# Autodesk Inventor assembly: 043(F,D-166-3)
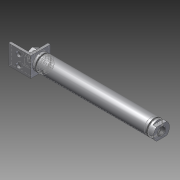
[picture p0: Inventor's stored thumbnail of the model, 180x180]
Saved by Autodesk Inventor 2012 (Build 160160000, 160)
## iProperties
Category: PARTsolutions
Company: BIMBA
Created: 2013-01-17
Part Number: 043(F,D-166-3)
Catalog Web Link: www.cadenas.de
Description: Original Line Standard Air Cylinders-
Vendor: BIMBA
Document SubType Name: Assembly
Designer: William
Manufacturer: BIMBA
PSOL_IDENT_0: {\\10.0.0.242\data_v9\23d-libs\bimba\bimba\bimba_imperial\bimba_full_line\original_line_cylinders\st
PSOL_IDENT_1: andard_air_cylinders\standard_air_cylinder_asmtab.prj},308 {VTYP=3D},{STYP=ASSTAB},{NB=043(F,D-166-3
PSOL_IDENT_2: )},{LINA=043},{NN=Original Line Standard Air Cylinders},{DATE=06.09.2012 11:26:56},{GEOMDATE=06.09.2
PSOL_IDENT_3: 012},{VERSION=},{LINEID=50},{LINESUBID=-1},{WBVAR=STROKE,ACTING,MNT,DER,NR,BM,CO,OO,VO,M,EE,EEL,K,Q,
PSOL_IDENT_4: Y,G,T,B,H,SER,SR,NT,W,HL,STPT1,STPT2,STPT3,STPT4,MB,PB,PRC,TB,MN}  {NB=043(F,D-166-3)},{LINA=043},{K
PSOL_IDENT_5: T=DUMMY},{PN=043},{PNC=043(F,D-166-3)},{PNA=(D-166-3)},{DASH=},{BORE1=0.75000000},{BORE=3/4\" (04)},
PSOL_IDENT_6: {BOREPN=04},{STROKE=3.000},{STROKEALG=[0.011:50/0.001]},{STROKE1=3.000},{ACTING=},{ACTINGALG= '' , '
PSOL_IDENT_7: Single Acting (SA)' , 'R' , 'Reverse Single Acting (SA)' , 'D' , 'Double Acting (SA)' },{ACTINGPN=},
PSOL_IDENT_8: {MNT=},{MNTALG= '' , 'Front Nose Mounting (SA)' , 'P' , 'Rear Pivot Mounting (SA)' , 'BF' , 'Front B
PSOL_IDENT_9: lock Mounting (SA)' , 'BR' , 'Rear Block Mounting for Vertical Positioning (SA)' , 'BFT' , 'Front Bl
PSOL_IDENT_10: ock Trunnion Mounting (SA)' , 'BRT' , 'Rear Block Trunnion Mounting (SA)' , 'A' , 'Double End Mounti
PSOL_IDENT_11: ng with Brackets and Adjustable Stroke (SA)' , 'AP' , 'Rear Pivot Mounting with Adjustable Stroke (S
PSOL_IDENT_12: A)' },{TYPE=},{MNTPN=},{DER=},{DERALG= '' , 'N/A' },{NR=},{NRALG= '' , 'Round (Standard)' , 'NR' , '
PSOL_IDENT_13: Non-rotating - Hexagon Rod' },{NRPN=},{BM=},{BMALG= '' , 'Without Built-in Midget 3-Way Solenoid Ope
PSOL_IDENT_14: rated Valve' , 'LS' , 'With LS Series Solenoid Valve [LS]' },{BMPN=},{CO=},{COALG= '' , 'N/A' },{OO=
PSOL_IDENT_15: },{OOALG= '', 'N/A' },{OOPN=},{VO=Z},{VOALG= 'Z' , 'N/A' },{VOPN=},{OOVOPN=},{M=},{MALG= '', 'Withou
PSOL_IDENT_16: t Magnet', 'M', 'With Magnet' },{EE=},{EEL=0.000},{EEMAX=47.0000},{EEALG= '', 'Without Extra Extensi
PSOL_IDENT_17: on', 'EE', 'With Extra Extension' },{EELALG=0},{EEPN=},{EEPN1=0.000},{K=},{KALG= '' , 'N/A' },{KPN=}
PSOL_IDENT_18: ,{Q=},{QALG= '' , 'Standard Port' , 'Q' , 'Side Port' },{QPN=},{Y=},{YALG= '' , 'N/A' },{YPN=},{YCON
PSOL_IDENT_19: =},{F=},{FALG= '', 'Non-Coated (Standard)', 'F', 'Molycoated' },{FPN=},{G=},{GPN=},{GPN99=},{T=},{TA
PSOL_IDENT_20: LG= '' , 'Standard -20° to 200°F (-29° to 95°C)' , 'N' , 'Low Temperature' , 'V' , 'High Temperature
PSOL_IDENT_21: ' },{NPN=},{VPN=},{B=},{BALG= '', 'W/out Bumpers' , 'B' , 'W/ Bumpers' },{BPN=},{H=},{HALG= '', 'W/
PSOL_IDENT_22: Standard Spring (Relaxed 3 lbs./Compressed 6 lbs.)', 'H', 'W/ Heavy Spring (Relaxed 4 lbs./Compresse
PSOL_IDENT_23: d 10 lbs.)' },{HPN=},{SER=},{SERALG= '' , 'N/A' },{SR=C},{SRALG= 'C' , 'Standard Blackened Carbon St
PSOL_IDENT_24: eel' , 'SR' , 'Stainless Steel [SR]' },{SRPN=},{SRCON=1},{NT=},{NTPN=},{W=},{WALG= '' , 'N/A' },{WPN
PSOL_IDENT_25: =},{E=},{EALG= '' , 'Standard Seals/Lube' , 'E' , 'Non-Lube Seals/Lube' },{EPN=},{HL=},{HLALG= '' ,
PSOL_IDENT_26: 'N/A' },{ST=},{STALG= '' , 'N/A' },{STPT1=},{STPT1ALG= '' , 'N/A' },{STPT2=},{STPT2ALG= '' , 'N/A' }
PSOL_IDENT_27: ,{STPT3=},{STPT3ALG= '' , 'N/A' },{STPT4=},{STPT4ALG= '' , 'N/A' },{STPN=},{MB=},{MBALG= '' , 'Witho
PSOL_IDENT_28: ut Mounting Bracket' , 'F,D-226' , 'D-226 (front)' },{MBPN=},{MBPNALL=D-226},{MBPNALLREAR=},{PB=},{P
PSOL_IDENT_29: BALG= '' , 'N/A' },{PBPN=},{PBPNALL=},{PRC=F,D-166-3},{PRCALG= '' , 'W/out Pivot Rod Clevis' , 'F,D-
PSOL_IDENT_30: 166-3' , 'D-166-3 (front)' },{PRCPN=(F,D-166-3)},{PRCPNALL=D-166-3},{TB=},{TBALG= '' , 'N/A' },{TBPN
PSOL_IDENT_31: =},{TBPNALL=},{MN=},{MNALG= '' , 'N/A' },{MNPN=},{MNCONF=},{MNCONR=},{TLEN=5.6360},{FRAC=7.2600},{RG
PSOL_IDENT_32: CON=},{RGDACCON=},{RHCON=},{RHCON1=},{RHCONON=1},{RHACCON=},{FNUTCON=1},{RNUTCON=0},{FNUTPN=D-98},{R
PSOL_IDENT_33: NUTPN=},{FNUTTRANS=0.0000},{RNUTTRANS=0.0000},{VHOLECON=2},{A1=0.8750},{A1N=0.8750},{A1P=1.5940},{A1
PSOL_IDENT_34: B=1.5940},{A4=0.3130},{A4N=0.3130},{A4P=0.2525},{A5=0.0300},{A1H=0.531},{A1NH=0.5310},{A1PH=1.5940},
PSOL_IDENT_35: {A1BH=1.0940},{A1SH=1.2190},{A2H=0.2190},{A2NH=0.2190},{LENGTH=1.5000},{LENGTH1=1.5000},{LENGTH2=3.0
PSOL_IDENT_36: 300},{MUL=5.0700},{MUL11=5.0700},{MUL22=8.07},{MUL33=5.0700},{MUL2=1.6900},{MUL211=1.6900},{MUL222=2
PSOL_IDENT_37: .6900},{MUL233=1.6900},{SSS=6.0000},{RGLEN=0.5920},{RHLEN=0.3420},{SSS1=4.0000},{A13=1.3120},{DIF=0.
PSOL_IDENT_38: 0000},{G5=0.6250},{ON=0},{SSADD=0.0000},{BADD=0.0000},{MADD=0.0000},{NVADD=0.0000},{TRACKL=5.3460},{
PSOL_IDENT_39: TRACKCON=D-74168},{TRIMCON=0},{TRIMCON1=0},{PINCON=},{FSPACE=0.6000},{SPACE=0.0750},{TEXT=0.1312},{S
PSOL_IDENT_40: 1=1.0000},{D1=0.8050},{D1N=0.8050},{D1B=0.8625},{D1P=0.8325},{FA=0.750},{RA=0.0000},{PPATH=standard_
PSOL_IDENT_41: air_cylinder_asmtpl.prj},{MATALGHTML=<b>Standard Original Line:</b><dl><dt>Rod:</dt><dd>- Stainless
PSOL_IDENT_42: Steel</dd><dd>&nbsp;&nbsp;(5/16  9/16 Bores)</dd><dd>- High Strength Carbon Steel</dd><dd>&nbsp;&nb
PSOL_IDENT_43: sp;(3/4  3 Bore)</dd><dd>- Stainless Steel</dd><dd>&nbsp;&nbsp;(X style DXP/DX/DXDE)</dd><dt>Bea
PSOL_IDENT_44: rings:</dt><dd>- Sintered Bronze</dd><dt>Body:</dt><dd>- 304 Stainless Steel</dd><dt>End Caps:</dt><
PSOL_IDENT_45: dd>- Aluminum</dd><dt>Seals:</dt><dd>- Buna N</dd></dl>},{ASSCFGPRA=04},{MBPNA=},{MNPNA=},{PRCPNA=(D
PSOL_IDENT_46: -166-3)},{ASSOPTACC=STPT4},{A=6.57},{HADD=0.0000},{WFL=0.25},{QADD=0.000},{QADD1=0.440},{TEST=3.0000
PSOL_IDENT_47: },{MNTB=},{STDNUTF=1},{STDNUTR=0}
CNS_NT: Standard Male Thread
CNS_NB: 043(F,D-166-3)
CNS_NBSYN: $PNC.
CNS_LINA: 043
CNS_PN: 043
CNS_PNC: 043(F,D-166-3)
CNS_PNA: (D-166-3)
CNS_BORE1: 0.75000000
CNS_BORE: 3/4" [04]
CNS_BOREPN: 04
CNS_STROKE: 3.000
CNS_STROKEALG: [0.011:50/0.001]
CNS_STROKE1: 3.000
CNS_ACTING: Standard Single
CNS_ACTINGALG: '' , 'Single Acting (SA)' , 'R' , 'Reverse Single Acting (SA)' , 'D' , 'Double Acting (SA)'
CNS_MNT: Standard Front Nose
CNS_MNTALG: '' , 'Front Nose Mounting (SA)' , 'P' , 'Rear Pivot Mounting (SA)' , 'BF' , 'Front Block Mounting (SA)' , 'BR' , 'Rear Block Mounting for Vertical Positioning (SA)' , 'BFT' , 'Front Block Trunnion Mounting (SA)' , 'BRT' , 'Rear Block Trunnion Mounting (SA)' , 'A' , 'Double End Mounting with Brackets and Adjustable Stroke (SA)' , 'AP' , 'Rear Pivot Mounting with Adjustable Stroke (SA)'
CNS_DER: N/A
CNS_DERALG: '' , 'N/A'
CNS_NR: Standard Round
CNS_NRALG: '' , 'Round (Standard)' , 'NR' , 'Non-rotating - Hexagon Rod'
CNS_BM: Without Solenoid Operated Valve
CNS_BMALG: '' , 'Without Built-in Midget 3-Way Solenoid Operated Valve' , 'LS' , 'With LS Series Solenoid Valve [LS]'
CNS_CO: N/A
CNS_COALG: '' , 'N/A'
CNS_OO: N/A
CNS_OOALG: '', 'N/A'
CNS_VO: N/A
CNS_VOALG: 'Z' , 'N/A'
CNS_M: Without Magnet Piston
CNS_MALG: '', 'Without Magnet', 'M', 'With Magnet'
CNS_EE: Standard Rod Extension
CNS_EEL: 0.000
CNS_EEMAX: 47.0000
CNS_EEALG: '', 'Without Extra Extension', 'EE', 'With Extra Extension'
CNS_EELALG: 0
CNS_EEPN1: 0.000
CNS_K: N/A
CNS_KALG: '' , 'N/A'
CNS_Q: Standard Axial Port
CNS_QALG: '' , 'Standard Port' , 'Q' , 'Side Port'
CNS_Y: N/A
CNS_YALG: '' , 'N/A'
CNS_FALG: '', 'Non-Coated (Standard)', 'F', 'Molycoated'
CNS_G: Standard Grease Lube
CNS_T: Standard -20° to 200°F (-29° to 95°C)
CNS_TALG: '' , 'Standard -20° to 200°F (-29° to 95°C)' , 'N' , 'Low Temperature' , 'V' , 'High Temperature'
CNS_B: Without Bumpers
CNS_BALG: '', 'W/out Bumpers' , 'B' , 'W/ Bumpers'
CNS_H: Standard (3 - 6 lbs.)
CNS_HALG: '', 'W/ Standard Spring (Relaxed 3 lbs./Compressed 6 lbs.)', 'H', 'W/ Heavy Spring (Relaxed 4 lbs./Compressed 10 lbs.)'
CNS_SER: N/A
CNS_SERALG: '' , 'N/A'
CNS_SR: Standard Blackened Carbon Steel
CNS_SRALG: 'C' , 'Standard Blackened Carbon Steel' , 'SR' , 'Stainless Steel [SR]'
CNS_SRCON: 1
CNS_W: N/A
CNS_WALG: '' , 'N/A'
CNS_EALG: '' , 'Standard Seals/Lube' , 'E' , 'Non-Lube Seals/Lube'
CNS_HL: N/A
CNS_HLALG: '' , 'N/A'
CNS_STALG: '' , 'N/A'
CNS_STPT1: N/A
CNS_STPT1ALG: '' , 'N/A'
CNS_STPT2: N/A
CNS_STPT2ALG: '' , 'N/A'
CNS_STPT3: N/A
CNS_STPT3ALG: '' , 'N/A'
CNS_STPT4: N/A
CNS_STPT4ALG: '' , 'N/A'
CNS_MB: Without Mounting Bracket
CNS_MBALG: '' , 'Without Mounting Bracket' , 'F,D-226' , 'D-226 (front)'
CNS_MBPNALL: D-226
CNS_PB: N/A
CNS_PBALG: '' , 'N/A'
CNS_PRC: D-166-3 (front)
CNS_PRCALG: '' , 'W/out Pivot Rod Clevis' , 'F,D-166-3' , 'D-166-3 (front)'
CNS_PRCPN: (F,D-166-3)
CNS_PRCPNALL: D-166-3
CNS_TB: N/A
CNS_TBALG: '' , 'N/A'
CNS_MN: N/A
CNS_MNALG: '' , 'N/A'
CNS_TLEN: 5.6360
CNS_FRAC: 7.2600
CNS_RHCONON: 1
CNS_FNUTCON: 1
CNS_RNUTCON: 0
CNS_FNUTPN: D-98
CNS_FNUTTRANS: 0.0000
CNS_RNUTTRANS: 0.0000
CNS_VHOLECON: 2
CNS_A1: 0.8750
CNS_A1N: 0.8750
CNS_A1P: 1.5940
CNS_A1B: 1.5940
CNS_A4: 0.3130
CNS_A4N: 0.3130
CNS_A4P: 0.2525
CNS_A5: 0.0300
CNS_A1H: 0.531
CNS_A1NH: 0.5310
CNS_A1PH: 1.5940
CNS_A1BH: 1.0940
CNS_A1SH: 1.2190
CNS_A2H: 0.2190
CNS_A2NH: 0.2190
CNS_LENGTH: 1.5000
CNS_LENGTH1: 1.5000
CNS_LENGTH2: 3.0300
CNS_MUL: 5.0700
CNS_MUL11: 5.0700
CNS_MUL22: 8.070
CNS_MUL33: 5.0700
CNS_MUL2: 1.6900
CNS_MUL211: 1.6900
CNS_MUL222: 2.6900
CNS_MUL233: 1.6900
CNS_SSS: 6.0000
CNS_RGLEN: 0.5920
CNS_RHLEN: 0.3420
CNS_SSS1: 4.0000
CNS_A13: 1.3120
CNS_DIF: 0.0000
CNS_G5: 0.6250
CNS_ON: 0
CNS_SSADD: 0.0000
CNS_BADD: 0.0000
CNS_MADD: 0.0000
CNS_NVADD: 0.0000
CNS_TRACKL: 5.3460
CNS_TRACKCON: D-74168
CNS_TRIMCON: 0
CNS_TRIMCON1: 0
CNS_FSPACE: 0.6000
CNS_SPACE: 0.0750
CNS_TEXT: 0.1312
CNS_S1: 1.0000
CNS_D1: 0.8050
CNS_D1N: 0.8050
CNS_D1B: 0.8625
CNS_D1P: 0.8325
CNS_FA: 0.750
CNS_RA: 0.0000
CNS_PPATH: standard_air_cylinder_asmtpl.prj
CNS_MATALGHTML: <b>Standard Original Line:</b><dl><dt>Rod:</dt><dd>- Stainless Steel</dd><dd>&nbsp;&nbsp;(5/16  9/16 Bores)</dd><dd>- High Strength Carbon Steel</dd><dd>&nbsp;&nbsp;(3/4  3 Bore)</dd><dd>- Stainless Steel</dd><dd>&nbsp;&nbsp;(X style DXP/DX/DXDE)</dd><dt>Bearings:</dt><dd>- Sintered Bronze</dd><dt>Body:</dt><dd>- 304 Stainless Steel</dd><dt>End Caps:</dt><dd>- Aluminum</dd><dt>Seals:</dt><dd>- Buna N</dd></dl>
CNS_ASSCFGPRA: 04
CNS_PRCPNA: (D-166-3)
CNS_ASSOPTACC: STPT4
CNS_A: 6.57
CNS_HADD: 0.0000
CNS_WFL: 0.250
CNS_QADD: 0.000
CNS_QADD1: 0.440
CNS_TEST: 3.0000
CNS_STDNUTF: 1
CNS_STDNUTR: 0
SUPPLIER: BIMBA
ARTICLENO: 043(F,D-166-3)
BOMINFO: 043
CREATOR: CADENAS GmbH
Title: 043
Author: Cadenas PARTsolutions
## Documents named in this file (7)
- C:\Users\William\Desktop\FRC CAD Files\Robot2013\Launcher\Piston\.75 inch\043(F,D-166-3).iam
- C:\Users\William\Desktop\FRC CAD Files\Robot2013\Launcher\Piston\.75 inch\04000_rod_guide.ipt
- C:\Users\William\Desktop\FRC CAD Files\Robot2013\Launcher\Piston\.75 inch\D-166-3-dummy.ipt
- C:\Users\William\Desktop\FRC CAD Files\Robot2013\Launcher\Piston\.75 inch\04-5_6362C.ipt
- C:\Users\William\Desktop\FRC CAD Files\Robot2013\Launcher\Piston\.75 inch\040000_rear_head.ipt
- C:\Users\William\Desktop\FRC CAD Files\Robot2013\Launcher\Piston\.75 inch\D-98.ipt
- C:\Users\William\Desktop\FRC CAD Files\Robot2013\Launcher\Piston\.75 inch\Piston Mounting Bracket.ipt
## Components (6 placed, 6 different names)
1. 04000_rod_guide:1 — to_tube_XY@1 <-> tube_front_XY@9, to_tube_Z@1 <-> tube_front_Z@9, to_tube_YZ@1 <-> tube_front_YZ@9, Mate:14, Mate:15, Mate:17
2. D-166-3-dummy:1
3. 04-5_6362C:1 — to_tube_XY@1 <-> tube_front_XY@9, to_tube_Z@1 <-> tube_front_Z@9, to_tube_YZ@1 <-> tube_front_YZ@9, tube_rear_XY@9 <-> to_tube_XY@10, tube_rear_Z@9 <-> to_tube_Z@10, tube_rear_YZ@9 <-> to_tube_YZ@10
4. 040000_rear_head:1 — tube_rear_XY@9 <-> to_tube_XY@10, tube_rear_Z@9 <-> to_tube_Z@10, tube_rear_YZ@9 <-> to_tube_YZ@10, Angle:5
5. D-98:1 — Mate:16, Mate:17, Angle:4, Angle:5
6. Piston Mounting Bracket:1 — Mate:14, Mate:15, Mate:16, Angle:4
## Relationships (12: Mate 6, Angle 4, Flush 2)
- to_tube_XY@1 <-> tube_front_XY@9 [Flush]: 04000_rod_guide:1 ↔ 04-5_6362C:1
- to_tube_Z@1 <-> tube_front_Z@9 [Mate]: 04000_rod_guide:1 ↔ 04-5_6362C:1
- to_tube_YZ@1 <-> tube_front_YZ@9 [Angle] (0 deg): 04000_rod_guide:1 ↔ 04-5_6362C:1
- tube_rear_XY@9 <-> to_tube_XY@10 [Flush]: 04-5_6362C:1 ↔ 040000_rear_head:1
- tube_rear_Z@9 <-> to_tube_Z@10 [Mate]: 04-5_6362C:1 ↔ 040000_rear_head:1
- tube_rear_YZ@9 <-> to_tube_YZ@10 [Angle] (0 deg): 04-5_6362C:1 ↔ 040000_rear_head:1
- Mate:14: 04000_rod_guide:1 ↔ Piston Mounting Bracket:1
- Mate:15: 04000_rod_guide:1 ↔ Piston Mounting Bracket:1
- Mate:16: D-98:1 ↔ Piston Mounting Bracket:1
- Mate:17: 04000_rod_guide:1 ↔ D-98:1
- Angle:4 (30 deg): D-98:1 ↔ Piston Mounting Bracket:1
- Angle:5 (30 deg): 040000_rear_head:1 ↔ D-98:1
